# Autodesk Inventor assembly: ideal_diode_enclosure
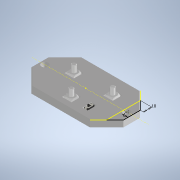
[picture p0: Inventor's stored thumbnail of the model, 180x180]
Saved by Autodesk Inventor 2021 (Build 250183000, 183)
## iProperties
Created: 2021-01-31
Part Number: ideal_diode_enclosure
Document SubType Name: Assembly
Designer: oskar
Author: oskar
## Documents named in this file (3)
- C:\Users\oskar\Dropbox\Dokument\Projekt\Elita\Electrical system\Highside-Powerdistribution\hardware\ideal-diode\cad\ideal_diode_enclosure.iam
- C:\Users\oskar\Dropbox\Dokument\Projekt\Elita\Electrical system\Highside-Powerdistribution\hardware\ideal-diode\cad\ideal_diode_ideal-diode.iam
- C:\Users\oskar\Dropbox\Dokument\Projekt\Elita\Electrical system\Highside-Powerdistribution\hardware\ideal-diode\cad\ideal_diode_enclosure.ipt
## Components (2 placed, 2 different names)
1. ideal_diode_ideal-diode:1 [sub-assembly] — Flush:1
2. ideal_diode_enclosure:1 — Flush:1
## Relationships (1: Flush 1)
- Flush:1: ideal_diode_ideal-diode:1 ↔ ideal_diode_enclosure:1
